# Autodesk Inventor assembly: S2_zplate-assembly
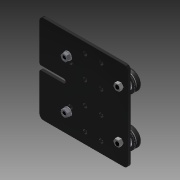
[picture p0: Inventor's stored thumbnail of the model, 180x180]
Saved by Autodesk Inventor 2014 (Build 180170000, 170)
## iProperties
Created: 2013-02-23
Part Number: S2_zplate-assembly
Document SubType Name: Assembly
Designer: Edward
Description: Spindle Mount Plate
Mass: 330.508 g
Surface Area: 462.689 cm^2
Volume: 52.0666 cm^3
Density: 6.34779 g/cm^3
Author: Edward
## Documents named in this file (7)
- C:\Users\Edward\Desktop\Shapeoko_v2.0\S2_zplate-assembly.iam
- C:\Users\Edward\Desktop\Shapeoko_v2.0\S2_Zplate.ipt
- C:\Users\Edward\Desktop\Shapeoko_v2.0\B18033.ipt
- C:\Users\Edward\Desktop\Shapeoko_v2.0\SM-H03.ipt
- C:\Users\Edward\Desktop\Shapeoko_v2.0\91239A233.ipt
- C:\Users\Edward\Desktop\Shapeoko_v2.0\SM-H04.ipt
- C:\Users\Edward\Desktop\Shapeoko_v2.0\B30037.iam
## Components (19 placed, 6 different names)
1. S2_Zplate:1 — Insert:5, Insert:6, Mate:2, Mate:4, Insert:9, Insert:10, Insert:16, Insert:18
2. B18033:1 — Insert:5, Mate:1
3. B18033:2 — Insert:6, Mate:3
4. SM-H03:2 — Mate:3, Mate:4, Insert:24
5. SM-H03:4 — Insert:9, Insert:23
6. SM-H03:5 — Mate:1, Mate:2, Insert:19
7. SM-H03:6 — Insert:10, Insert:21
8. SM-H03:7 — Insert:17, Insert:18
9. SM-H04:1 — Insert:17
10. SM-H03:8 — Insert:15, Insert:16
11. SM-H04:2 — Insert:15
12. 91239A233:5 — Insert:22
13. B30037:5 [sub-assembly] — Insert:21, Insert:22
14. B30037:6 [sub-assembly] — Insert:19, Insert:20
15. 91239A233:6 — Insert:20
16. 91239A233:7 — Insert:25
17. B30037:7 [sub-assembly] — Insert:23, Insert:26
18. B30037:8 [sub-assembly] — Insert:24, Insert:25
19. 91239A233:8 — Insert:26
## Relationships (20: Insert 16, Mate 4)
- Insert:5: S2_Zplate:1 ↔ B18033:1
- Insert:6: S2_Zplate:1 ↔ B18033:2
- Mate:1: B18033:1 ↔ SM-H03:5
- Mate:2: S2_Zplate:1 ↔ SM-H03:5
- Mate:3: B18033:2 ↔ SM-H03:2
- Mate:4: S2_Zplate:1 ↔ SM-H03:2
- Insert:9: S2_Zplate:1 ↔ SM-H03:4
- Insert:10: S2_Zplate:1 ↔ SM-H03:6
- Insert:15: SM-H03:8 ↔ SM-H04:2
- Insert:16: S2_Zplate:1 ↔ SM-H03:8
- Insert:17: SM-H03:7 ↔ SM-H04:1
- Insert:18: S2_Zplate:1 ↔ SM-H03:7
- Insert:19: SM-H03:5 ↔ B30037:6
- Insert:20: B30037:6 ↔ 91239A233:6
- Insert:21: SM-H03:6 ↔ B30037:5
- Insert:22: 91239A233:5 ↔ B30037:5
- Insert:23: SM-H03:4 ↔ B30037:7
- Insert:24: SM-H03:2 ↔ B30037:8
- Insert:25: 91239A233:7 ↔ B30037:8
- Insert:26: B30037:7 ↔ 91239A233:8
